# Autodesk Inventor assembly: Final2
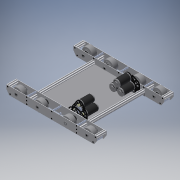
[picture p0: Inventor's stored thumbnail of the model, 180x180]
Saved by Autodesk Inventor 2016 (Build 200138000, 138)
## iProperties
Created: 2017-01-21
Part Number: Final2
Document SubType Name: Assembly
Designer: hamblettk
Author: hamblettk
## Documents named in this file (11)
- E:\1073CAD\Robot2017\DriveTrain\Final2.iam
- E:\1073CAD\Robot2017\DriveTrain\OutsidePlate2.ipt
- E:\1073CAD\Robot2017\DriveTrain\Individual Parts\3.625Churro.ipt
- E:\1073CAD\Robot2017\DriveTrain\Individual Parts\Mock 8020 3.375in.ipt
- E:\1073CAD\Robot2017\DriveTrain\InsidePlate2.ipt
- E:\1073CAD\Robot2017\DriveTrain\Individual Parts\Mock 8020 28.25in.ipt
- E:\1073CAD\Robot2017\DriveTrain\Individual Parts\DoublePulleyGearbox.iam
- E:\1073CAD\Robot2017\DriveTrain\Individual Parts\SinglePulley.iam
- E:\1073CAD\Robot2017\DriveTrain\Individual Parts\DoublePulley.iam
- E:\1073CAD\Robot2017\DriveTrain\Individual Parts\14-20Bolt.ipt
- E:\1073CAD\Robot2017\DriveTrain\BellyPan2.ipt
## Components (54 placed, 10 different names)
1. OutsidePlate2:1 — Mate:1, Mate:2, Mate:3, Mate:4, Mate:5, Mate:6, Mate:7, Mate:8, Mate:9, Mate:10, Flush:1, Flush:2, Mate:12, Mate:13, Mate:29, Mate:30, Mate:32, Mate:33, Mate:36, Mate:37, Mate:40, Mate:41, Mate:44, Mate:45, Mate:46, Mate:47, Mate:48, Mate:49, Mate:50, Mate:51, Mate:52, Mate:53, Mate:54, Mate:55, Mate:68, Mate:69, Mate:70, Mate:71, Mate:72, Mate:73, Mate:74, Mate:75, Mate:76, Mate:77, Mate:78, Mate:79
2. 3.625Churro:1 — Mate:1
3. 3.625Churro:2 — Mate:8
4. 3.625Churro:3 — Mate:7
5. 3.625Churro:4 — Mate:6
6. 3.625Churro:5 — Mate:4
7. 3.625Churro:6 — Mate:5
8. 3.625Churro:7 — Mate:2
9. 3.625Churro:8 — Mate:3
10. Mock 8020 3.375in:1 — Mate:9, Mate:11
11. Mock 8020 3.375in:2 — Mate:10
12. InsidePlate2:1 — Mate:11, Flush:1, Flush:2, Mate:31, Mate:90
13. Mock 8020 28.25in:1 — Mate:13, Mate:15, Mate:16, Mate:91, Flush:9
14. Mock 8020 28.25in:2 — Mate:12, Mate:14
15. OutsidePlate2:2 — Mate:14, Mate:15, Mate:16, Flush:3, Flush:4, Mate:25, Mate:26, Mate:27, Mate:42, Mate:43
16. InsidePlate2:2 — Flush:3, Flush:4, Mate:17, Mate:18, Mate:19, Mate:20, Mate:21, Mate:22, Mate:23, Mate:24, Mate:28, Mate:34, Mate:35, Mate:38, Mate:39, Mate:56, Mate:57, Flush:5, Flush:6, Flush:7, Flush:8, Mate:58, Mate:59, Mate:60, Mate:62, Mate:64, Mate:66, Mate:67, Mate:80, Mate:81, Mate:82, Mate:84, Mate:86, Mate:88, Mate:89
17. 3.625Churro:9 — Mate:17
18. 3.625Churro:10 — Mate:18
19. 3.625Churro:11 — Mate:19
20. 3.625Churro:12 — Mate:20, Mate:25
21. 3.625Churro:13 — Mate:21
22. 3.625Churro:14 — Mate:22
23. 3.625Churro:15 — Mate:23
24. 3.625Churro:16 — Mate:24
25. DoublePulleyGearbox:1 [sub-assembly] — Mate:29, Mate:30, Mate:31
26. DoublePulleyGearbox:2 [sub-assembly] — Mate:26, Mate:27, Mate:28
27. SinglePulley:1 [sub-assembly] — Mate:32, Mate:33
28. SinglePulley:2 [sub-assembly] — Mate:36, Mate:37
29. SinglePulley:3 [sub-assembly] — Mate:38, Mate:39
30. SinglePulley:4 [sub-assembly] — Mate:34, Mate:35
31. DoublePulley:1 [sub-assembly] — Mate:40, Mate:41
32. DoublePulley:2 [sub-assembly] — Mate:42, Mate:43
33. 14-20Bolt:1 — Mate:44, Mate:68
34. 14-20Bolt:2 — Mate:45, Mate:69
35. 14-20Bolt:3 — Mate:46, Mate:70
36. 14-20Bolt:4 — Mate:47, Mate:71
37. 14-20Bolt:5 — Mate:48, Mate:72
38. 14-20Bolt:6 — Mate:49, Mate:73
39. 14-20Bolt:7 — Mate:50, Mate:74
40. 14-20Bolt:8 — Mate:51, Mate:75
41. 14-20Bolt:9 — Mate:54, Mate:79
42. 14-20Bolt:10 — Mate:55, Mate:78
43. 14-20Bolt:11 — Mate:52, Mate:76
44. 14-20Bolt:12 — Mate:53, Mate:77
45. 14-20Bolt:13 — Mate:66, Mate:88
46. 14-20Bolt:14 — Mate:67, Mate:89
47. 14-20Bolt:15 — Mate:64, Mate:86
48. 14-20Bolt:17 — Mate:62, Mate:84
49. 14-20Bolt:19 — Mate:60, Mate:82
50. 14-20Bolt:21 — Mate:58, Mate:80
51. 14-20Bolt:22 — Mate:59, Mate:81
52. Mock 8020 3.375in:3 — Mate:56, Flush:7, Flush:8
53. Mock 8020 3.375in:4 — Mate:57, Flush:5, Flush:6
54. BellyPan2:1 — Mate:90, Mate:91, Flush:9
## Relationships (94: Mate 85, Flush 9)
- Mate:1: OutsidePlate2:1 ↔ 3.625Churro:1
- Mate:2: OutsidePlate2:1 ↔ 3.625Churro:7
- Mate:3: OutsidePlate2:1 ↔ 3.625Churro:8
- Mate:4: OutsidePlate2:1 ↔ 3.625Churro:5
- Mate:5: OutsidePlate2:1 ↔ 3.625Churro:6
- Mate:6: OutsidePlate2:1 ↔ 3.625Churro:4
- Mate:7: OutsidePlate2:1 ↔ 3.625Churro:3
- Mate:8: OutsidePlate2:1 ↔ 3.625Churro:2
- Mate:9: OutsidePlate2:1 ↔ Mock 8020 3.375in:1
- Mate:10: OutsidePlate2:1 ↔ Mock 8020 3.375in:2
- Mate:11: Mock 8020 3.375in:1 ↔ InsidePlate2:1
- Flush:1: OutsidePlate2:1 ↔ InsidePlate2:1
- Flush:2: OutsidePlate2:1 ↔ InsidePlate2:1
- Mate:12: OutsidePlate2:1 ↔ Mock 8020 28.25in:2
- Mate:13: OutsidePlate2:1 ↔ Mock 8020 28.25in:1
- Mate:14: Mock 8020 28.25in:2 ↔ OutsidePlate2:2
- Mate:15: Mock 8020 28.25in:1 ↔ OutsidePlate2:2
- Mate:16: Mock 8020 28.25in:1 ↔ OutsidePlate2:2
- Flush:3: OutsidePlate2:2 ↔ InsidePlate2:2
- Flush:4: OutsidePlate2:2 ↔ InsidePlate2:2
- Mate:17: InsidePlate2:2 ↔ 3.625Churro:9
- Mate:18: InsidePlate2:2 ↔ 3.625Churro:10
- Mate:19: InsidePlate2:2 ↔ 3.625Churro:11
- Mate:20: InsidePlate2:2 ↔ 3.625Churro:12
- Mate:21: InsidePlate2:2 ↔ 3.625Churro:13
- Mate:22: InsidePlate2:2 ↔ 3.625Churro:14
- Mate:23: InsidePlate2:2 ↔ 3.625Churro:15
- Mate:24: InsidePlate2:2 ↔ 3.625Churro:16
- Mate:25: OutsidePlate2:2 ↔ 3.625Churro:12
- Mate:26: OutsidePlate2:2 ↔ DoublePulleyGearbox:2
- Mate:27: OutsidePlate2:2 ↔ DoublePulleyGearbox:2
- Mate:28: InsidePlate2:2 ↔ DoublePulleyGearbox:2
- Mate:29: OutsidePlate2:1 ↔ DoublePulleyGearbox:1
- Mate:30: OutsidePlate2:1 ↔ DoublePulleyGearbox:1
- Mate:31: InsidePlate2:1 ↔ DoublePulleyGearbox:1
- Mate:32: OutsidePlate2:1 ↔ SinglePulley:1
- Mate:33: OutsidePlate2:1 ↔ SinglePulley:1
- Mate:34: InsidePlate2:2 ↔ SinglePulley:4
- Mate:35: InsidePlate2:2 ↔ SinglePulley:4
- Mate:36: OutsidePlate2:1 ↔ SinglePulley:2
- Mate:37: OutsidePlate2:1 ↔ SinglePulley:2
- Mate:38: InsidePlate2:2 ↔ SinglePulley:3
- Mate:39: InsidePlate2:2 ↔ SinglePulley:3
- Mate:40: OutsidePlate2:1 ↔ DoublePulley:1
- Mate:41: OutsidePlate2:1 ↔ DoublePulley:1
- Mate:42: OutsidePlate2:2 ↔ DoublePulley:2
- Mate:43: OutsidePlate2:2 ↔ DoublePulley:2
- Mate:44: OutsidePlate2:1 ↔ 14-20Bolt:1
- Mate:45: OutsidePlate2:1 ↔ 14-20Bolt:2
- Mate:46: OutsidePlate2:1 ↔ 14-20Bolt:3
- Mate:47: OutsidePlate2:1 ↔ 14-20Bolt:4
- Mate:48: OutsidePlate2:1 ↔ 14-20Bolt:5
- Mate:49: OutsidePlate2:1 ↔ 14-20Bolt:6
- Mate:50: OutsidePlate2:1 ↔ 14-20Bolt:7
- Mate:51: OutsidePlate2:1 ↔ 14-20Bolt:8
- Mate:52: OutsidePlate2:1 ↔ 14-20Bolt:11
- Mate:53: OutsidePlate2:1 ↔ 14-20Bolt:12
- Mate:54: OutsidePlate2:1 ↔ 14-20Bolt:9
- Mate:55: OutsidePlate2:1 ↔ 14-20Bolt:10
- Mate:56: InsidePlate2:2 ↔ Mock 8020 3.375in:3
- Mate:57: InsidePlate2:2 ↔ Mock 8020 3.375in:4
- Flush:5: InsidePlate2:2 ↔ Mock 8020 3.375in:4
- Flush:6: InsidePlate2:2 ↔ Mock 8020 3.375in:4
- Flush:7: InsidePlate2:2 ↔ Mock 8020 3.375in:3
- Flush:8: InsidePlate2:2 ↔ Mock 8020 3.375in:3
- Mate:58: InsidePlate2:2 ↔ 14-20Bolt:21
- Mate:59: InsidePlate2:2 ↔ 14-20Bolt:22
- Mate:60: InsidePlate2:2 ↔ 14-20Bolt:19
- Mate:62: InsidePlate2:2 ↔ 14-20Bolt:17
- Mate:64: InsidePlate2:2 ↔ 14-20Bolt:15
- Mate:66: InsidePlate2:2 ↔ 14-20Bolt:13
- Mate:67: InsidePlate2:2 ↔ 14-20Bolt:14
- Mate:68: OutsidePlate2:1 ↔ 14-20Bolt:1
- Mate:69: OutsidePlate2:1 ↔ 14-20Bolt:2
- Mate:70: OutsidePlate2:1 ↔ 14-20Bolt:3
- Mate:71: OutsidePlate2:1 ↔ 14-20Bolt:4
- Mate:72: OutsidePlate2:1 ↔ 14-20Bolt:5
- Mate:73: OutsidePlate2:1 ↔ 14-20Bolt:6
- Mate:74: OutsidePlate2:1 ↔ 14-20Bolt:7
- Mate:75: OutsidePlate2:1 ↔ 14-20Bolt:8
- Mate:76: OutsidePlate2:1 ↔ 14-20Bolt:11
- Mate:77: OutsidePlate2:1 ↔ 14-20Bolt:12
- Mate:78: OutsidePlate2:1 ↔ 14-20Bolt:10
- Mate:79: OutsidePlate2:1 ↔ 14-20Bolt:9
- Mate:80: InsidePlate2:2 ↔ 14-20Bolt:21
- Mate:81: InsidePlate2:2 ↔ 14-20Bolt:22
- Mate:82: InsidePlate2:2 ↔ 14-20Bolt:19
- Mate:84: InsidePlate2:2 ↔ 14-20Bolt:17
- Mate:86: InsidePlate2:2 ↔ 14-20Bolt:15
- Mate:88: InsidePlate2:2 ↔ 14-20Bolt:13
- Mate:89: InsidePlate2:2 ↔ 14-20Bolt:14
- Mate:90: InsidePlate2:1 ↔ BellyPan2:1
- Mate:91: Mock 8020 28.25in:1 ↔ BellyPan2:1
- Flush:9: Mock 8020 28.25in:1 ↔ BellyPan2:1
